# Autodesk Inventor assembly: World
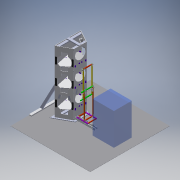
[picture p0: Inventor's stored thumbnail of the model, 180x180]
Saved by Autodesk Inventor 2019 (Build 230136000, 136)
## iProperties
Created: 2019-01-09
Part Number: World
Document SubType Name: Assembly
Designer: james
Author: james
## Documents named in this file (6)
- F:\JimsDesign\2019CHS4089\World.iam
- F:\JimsDesign\Library\Jims\Carpet.ipt
- F:\JimsDesign\2019CHS4089\FullSide.iam
- F:\JimsDesign\2019CHS4089\FullElevator.iam
- F:\JimsDesign\2019CHS4089\SizingCube.ipt
- F:\JimsDesign\FRCFeilds\2019\Team_Drawings_AllFiles\All Files\CADFiles\TE-19113\TE-19113.iam
## Components (5 placed, 5 different names)
1. Carpet:1 — Mate:1, Mate:3, Mate:5, Flush:1
2. FullSide:1 [sub-assembly] — Mate:1, Mate:6, Flush:2, Flush:3
3. FullElevator:1 [sub-assembly] — Mate:6, Flush:2, Flush:3
4. SizingCube:2 — Mate:3
5. TE-19113:1 [sub-assembly] — Mate:5, Flush:1
## Relationships (7: Mate 4, Flush 3)
- Mate:1 (35.56 mm): Carpet:1 ↔ FullSide:1
- Mate:3: Carpet:1 ↔ SizingCube:2
- Mate:5: Carpet:1 ↔ TE-19113:1
- Flush:1: Carpet:1 ↔ TE-19113:1
- Mate:6: FullSide:1 ↔ FullElevator:1
- Flush:2: FullSide:1 ↔ FullElevator:1
- Flush:3 (101.6 mm): FullSide:1 ↔ FullElevator:1
